# Autodesk Inventor assembly: F-wing
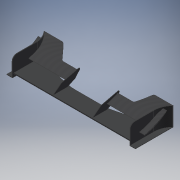
[picture p0: Inventor's stored thumbnail of the model, 180x180]
Saved by Autodesk Inventor 2018.1 (Build 221171000, 171)
## iProperties
Created: 2017-11-03
Part Number: F-wing
Material: 一般
Document SubType Name: Assembly
Designer: ku_sk
Mass: 6094.74 g
Surface Area: 13691.1 cm^2
Volume: 4262.05 cm^3
Density: 1.43 g/cm^3
Author: ku_sk
## Documents named in this file (6)
- D:\ku_sk\ドキュメント\Inventor\AeroCAD2018\CAD\Inventor\Aero Parts\F-wing\type7\F-wing.iam
- D:\ku_sk\ドキュメント\Inventor\AeroCAD2018\CAD\Inventor\Aero Parts\F-wing\type7\parts\type7_base.ipt
- D:\ku_sk\ドキュメント\Inventor\AeroCAD2018\CAD\Inventor\Aero Parts\F-wing\type7\parts\type7_end_plate.ipt
- D:\ku_sk\ドキュメント\Inventor\AeroCAD2018\CAD\Inventor\Aero Parts\F-wing\type7\parts\type7_end_plate_MIR.ipt
- D:\ku_sk\ドキュメント\Inventor\AeroCAD2018\CAD\Inventor\Aero Parts\F-wing\type7\parts\type7_element.ipt
- D:\ku_sk\ドキュメント\Inventor\AeroCAD2018\CAD\Inventor\Aero Parts\F-wing\type7\parts\type7_stay.ipt
## Components (6 placed, 5 different names)
1. type7_base:1 — フラッシュ:1, フラッシュ:2, フラッシュ:3, メイト:1, メイト:2, フラッシュ:4, メイト:3, メイト:8, メイト:9
2. type7_end_plate:1 — メイト:1, メイト:2, フラッシュ:4, フラッシュ:5, フラッシュ:6, メイト:4
3. type7_end_plate_MIR:1 — メイト:3, フラッシュ:5, フラッシュ:6, メイト:5
4. type7_element:1 — メイト:4, メイト:5, メイト:6, メイト:7
5. type7_stay:1 — メイト:6, メイト:8, フラッシュ:7
6. type7_stay:2 — メイト:7, メイト:9, フラッシュ:7
## Relationships (16: Mate 9, Flush 7)
- フラッシュ:1 [Flush]: type7_base:1
- フラッシュ:2 [Flush]: type7_base:1
- フラッシュ:3 [Flush]: type7_base:1
- メイト:1 [Mate]: type7_base:1 ↔ type7_end_plate:1
- メイト:2 [Mate]: type7_base:1 ↔ type7_end_plate:1
- フラッシュ:4 [Flush] (30 mm): type7_base:1 ↔ type7_end_plate:1
- メイト:3 [Mate]: type7_base:1 ↔ type7_end_plate_MIR:1
- フラッシュ:5 [Flush]: type7_end_plate:1 ↔ type7_end_plate_MIR:1
- フラッシュ:6 [Flush]: type7_end_plate:1 ↔ type7_end_plate_MIR:1
- メイト:4 [Mate]: type7_end_plate:1 ↔ type7_element:1
- メイト:5 [Mate]: type7_end_plate_MIR:1 ↔ type7_element:1
- メイト:6 [Mate]: type7_element:1 ↔ type7_stay:1
- メイト:7 [Mate]: type7_element:1 ↔ type7_stay:2
- メイト:8 [Mate]: type7_base:1 ↔ type7_stay:1
- メイト:9 [Mate]: type7_base:1 ↔ type7_stay:2
- フラッシュ:7 [Flush]: type7_stay:1 ↔ type7_stay:2
